# Autodesk Inventor assembly: Zespół7
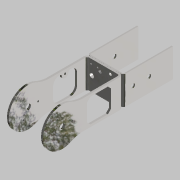
[picture p0: Inventor's stored thumbnail of the model, 180x180]
Saved by Autodesk Inventor 2021 (Build 250183000, 183)
## iProperties
Created: 2021-10-12
Part Number: Zespół7
Document SubType Name: Assembly
Designer: marci
Author: marci
## Documents named in this file (4)
- C:\Users\marci\Desktop\Projekt ramienia\3M2\Zespół7.iam
- C:\Users\marci\Desktop\Projekt ramienia\3M2\RR-PCSS-W3M2.ipt
- C:\Users\marci\Desktop\Projekt ramienia\3M2\RR-PCSS-W4M1D.1.ipt
- C:\Users\marci\Desktop\Projekt ramienia\3M2\RR-PCSS-W4M1D.2.ipt
## Components (3 placed, 3 different names)
1. RR-PCSS-W3M2:1 — Zestawiające:2, Równoległe:3, Równoległe:4
2. RR-PCSS-W4M1D.1:1 — Równoległe:1, Zestawiające:1, Równoległe:2, Zestawiające:2, Równoległe:4
3. RR-PCSS-W4M1D.2:1 — Równoległe:1, Zestawiające:1, Równoległe:2, Równoległe:3
## Relationships (6: Flush 4, Mate 2)
- Równoległe:1 [Flush]: RR-PCSS-W4M1D.1:1 ↔ RR-PCSS-W4M1D.2:1
- Zestawiające:1 [Mate]: RR-PCSS-W4M1D.1:1 ↔ RR-PCSS-W4M1D.2:1
- Równoległe:2 [Flush]: RR-PCSS-W4M1D.1:1 ↔ RR-PCSS-W4M1D.2:1
- Zestawiające:2 [Mate]: RR-PCSS-W3M2:1 ↔ RR-PCSS-W4M1D.1:1
- Równoległe:3 [Flush]: RR-PCSS-W3M2:1 ↔ RR-PCSS-W4M1D.2:1
- Równoległe:4 [Flush]: RR-PCSS-W3M2:1 ↔ RR-PCSS-W4M1D.1:1
